# Autodesk Inventor assembly: ASSY,MAIN,ELEVATOR
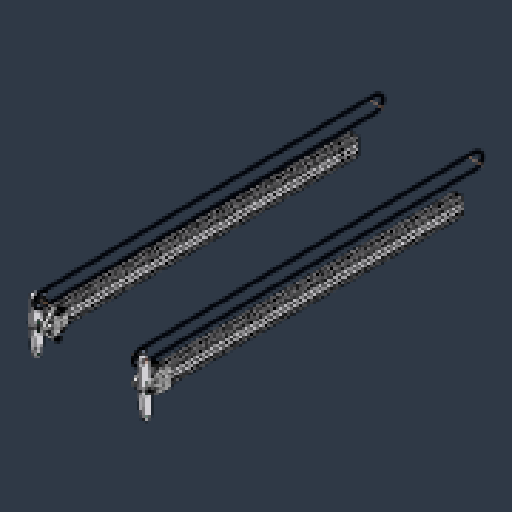
[picture p0: Inventor's stored thumbnail of the model, 512x512]
Saved by Autodesk Inventor 2024.3 (Build 283343000, 343)
## iProperties
Created: 2025-02-06
Part Number: ASSY,MAIN,ELEVATOR
Document SubType Name: Assembly
Designer: Jthib
Mfg Approved By: John.Thibert
Mass: 2913.72 g
Surface Area: 9344.89 cm^2
Volume: 863.068 cm^3
Density: 3.376 g/cm^3
ILogicPurgeVersion: 0.0.0.0
OnSaveVersion: 3.4.3.0
OnSaveAssembly: COREAutomationManager
ModelCat: Uncategorized
CN_MASS: 2.91
Author: Jthib
## Documents named in this file (12)
- C:\Users\Jthib\OneDrive\Robotics\4_Robot Files - 2025 - Poseidon\Elevator\ASSY,MAIN,ELEVATOR.iam
- C:\Users\Jthib\OneDrive\Robotics\4_Robot Files - 2025 - Poseidon\Elevator\SLIDE,TOP,ELEVATOR,STAGE1,LH.iam
- C:\Users\Jthib\OneDrive\Robotics\4_Robot Files - 2025 - Poseidon\Elevator\TUBE,MAIN,ELEVATOR,MAXTube-2x1-Holes.ipt
- C:\Users\Jthib\OneDrive\Robotics\4_Robot Files - 2025 - Poseidon\Chassis\PLUG,MAXTUBE,2IN,3DP.ipt
- C:\Users\Jthib\OneDrive\Robotics\4_Robot Files - 2025 - Poseidon\Elevator\PLUG,MAXTUBE,2IN,3DP,TOP,ELEVATOR.ipt
- C:\Users\Jthib\OneDrive\Robotics\4_Robot Files - 2025 - Poseidon\Elevator\PLATE,SIDE,PULLEY,MOUNT,TOP,ELEVATOR.ipt
- C:\Users\Jthib\OneDrive\Robotics\4_Robot Files - 2025 - Poseidon\Elevator\PLATE,ROCKER,ELEVATOR.ipt
- C:\Users\Jthib\OneDrive\Robotics\4_Robot Files - 2025 - Poseidon\Purchased\6663K11_ANSI Roller Chain Idler Sprocket\6663K11_ANSI Roller Chain Idler Sprocket\6663K11_ANSI Roller Chain Idler Sprocket.ipt
- C:\Users\Jthib\OneDrive\Robotics\4_Robot Files - 2025 - Poseidon\Chassis\#Poseidon 2025\Design Accelerator\Chain Drive2.iam
- C:\Users\Jthib\OneDrive\Robotics\4_Robot Files - 2025 - Poseidon\Elevator\SPACER,ROCKER,ELEVATOR.ipt
- C:\Users\Jthib\OneDrive\Robotics\4_Robot Files - 2025 - Poseidon\Fasteners\91259A585_NO THREADS_Alloy Steel Shoulder Screw\91259A585_NO THREADS_Alloy Steel Shoulder Screw\91259A585_NO THREADS_Alloy Steel Should.ipt
- C:\Users\Jthib\OneDrive\Robotics\4_Robot Files - 2025 - Poseidon\Elevator\SLIDE,TOP,ELEVATOR,STAGE1.iam
## Components (20 placed, 11 different names)
1. 6663K11_ANSI Roller Chain Idler Sprocket.ipt:1 — Mate:46
2. 6663K11_ANSI Roller Chain Idler Sprocket.ipt:2 — Mate:45
3. 91259A585_NO THREADS_Alloy Steel Should.ipt:1
4. 91259A585_NO THREADS_Alloy Steel Should.ipt:2
5. Chain Drive2.iam:1 [sub-assembly] — Mate:43, Mate:44
6. Chain Drive2.iam:2 [sub-assembly] — Mate:44
7. PLATE,ROCKER,ELEVATOR.ipt:1 — Mate:43, Mate:46
8. PLATE,ROCKER,ELEVATOR.ipt:2 — Mate:45
9. PLATE,SIDE,PULLEY,MOUNT,TOP,ELEVATOR.ipt:1
10. PLATE,SIDE,PULLEY,MOUNT,TOP,ELEVATOR.ipt:2 — Angle:3
11. PLUG,MAXTUBE,2IN,3DP,TOP,ELEVATOR.ipt:1
12. PLUG,MAXTUBE,2IN,3DP,TOP,ELEVATOR.ipt:2
13. PLUG,MAXTUBE,2IN,3DP.ipt:1 — Mate:42
14. PLUG,MAXTUBE,2IN,3DP.ipt:2 — Mate:41
15. SLIDE,TOP,ELEVATOR,STAGE1,LH.iam:1 [sub-assembly]
16. SLIDE,TOP,ELEVATOR,STAGE1.iam:1 [sub-assembly]
17. SPACER,ROCKER,ELEVATOR.ipt:1
18. SPACER,ROCKER,ELEVATOR.ipt:2
19. TUBE,MAIN,ELEVATOR,MAXTube-2x1-Holes.ipt:1 — Mate:39, Flush:5
20. TUBE,MAIN,ELEVATOR,MAXTube-2x1-Holes.ipt:2 — Angle:3, Flush:4, Mate:40
## Relationships (54: Mate 46, Flush 5, Angle 3)
- [Flush]: PLUG,MAXTUBE,2IN,3DP.ipt:1 ↔ TUBE,MAIN,ELEVATOR,MAXTube-2x1-Holes.ipt:1
- [Mate]: PLUG,MAXTUBE,2IN,3DP.ipt:1 ↔ TUBE,MAIN,ELEVATOR,MAXTube-2x1-Holes.ipt:1
- [Angle] (0 deg): PLUG,MAXTUBE,2IN,3DP.ipt:1 ↔ TUBE,MAIN,ELEVATOR,MAXTube-2x1-Holes.ipt:1
- [Mate]: SLIDE,TOP,ELEVATOR,STAGE1,LH.iam:1 ↔ TUBE,MAIN,ELEVATOR,MAXTube-2x1-Holes.ipt:1
- [Mate]: SLIDE,TOP,ELEVATOR,STAGE1,LH.iam:1 ↔ TUBE,MAIN,ELEVATOR,MAXTube-2x1-Holes.ipt:1
- [Mate]: SLIDE,TOP,ELEVATOR,STAGE1,LH.iam:1 ↔ TUBE,MAIN,ELEVATOR,MAXTube-2x1-Holes.ipt:1
- [Mate]: PLUG,MAXTUBE,2IN,3DP,TOP,ELEVATOR.ipt:1 ↔ TUBE,MAIN,ELEVATOR,MAXTube-2x1-Holes.ipt:1
- [Mate]: PLATE,SIDE,PULLEY,MOUNT,TOP,ELEVATOR.ipt:1 ↔ TUBE,MAIN,ELEVATOR,MAXTube-2x1-Holes.ipt:1
- [Mate]: PLATE,SIDE,PULLEY,MOUNT,TOP,ELEVATOR.ipt:1 ↔ PLUG,MAXTUBE,2IN,3DP,TOP,ELEVATOR.ipt:1
- [Mate]: PLATE,SIDE,PULLEY,MOUNT,TOP,ELEVATOR.ipt:1 ↔ PLUG,MAXTUBE,2IN,3DP,TOP,ELEVATOR.ipt:1
- [Mate]: PLATE,ROCKER,ELEVATOR.ipt:1 ↔ PLATE,SIDE,PULLEY,MOUNT,TOP,ELEVATOR.ipt:1
- [Mate]: PLATE,ROCKER,ELEVATOR.ipt:1 ↔ PLATE,SIDE,PULLEY,MOUNT,TOP,ELEVATOR.ipt:1
- [Mate]: PLATE,SIDE,PULLEY,MOUNT,TOP,ELEVATOR.ipt:1 ↔ TUBE,MAIN,ELEVATOR,MAXTube-2x1-Holes.ipt:1
- [Mate]: PLUG,MAXTUBE,2IN,3DP,TOP,ELEVATOR.ipt:1 ↔ TUBE,MAIN,ELEVATOR,MAXTube-2x1-Holes.ipt:1
- [Mate]: 6663K11_ANSI Roller Chain Idler Sprocket.ipt:1 ↔ Chain Drive2.iam:1
- [Mate] (0.1905 mm): 6663K11_ANSI Roller Chain Idler Sprocket.ipt:1 ↔ Chain Drive2.iam:1
- [Mate]: 91259A585_NO THREADS_Alloy Steel Should.ipt:1 ↔ SPACER,ROCKER,ELEVATOR.ipt:1
- [Mate]: 91259A585_NO THREADS_Alloy Steel Should.ipt:1 ↔ PLATE,SIDE,PULLEY,MOUNT,TOP,ELEVATOR.ipt:1
- [Mate]: 91259A585_NO THREADS_Alloy Steel Should.ipt:1 ↔ PLATE,ROCKER,ELEVATOR.ipt:1
- [Mate]: PLATE,ROCKER,ELEVATOR.ipt:1 ↔ SPACER,ROCKER,ELEVATOR.ipt:1
- [Flush]: PLUG,MAXTUBE,2IN,3DP.ipt:2 ↔ TUBE,MAIN,ELEVATOR,MAXTube-2x1-Holes.ipt:2
- [Mate]: PLUG,MAXTUBE,2IN,3DP.ipt:2 ↔ TUBE,MAIN,ELEVATOR,MAXTube-2x1-Holes.ipt:2
- [Angle] (0 deg): PLUG,MAXTUBE,2IN,3DP.ipt:2 ↔ TUBE,MAIN,ELEVATOR,MAXTube-2x1-Holes.ipt:2
- [Mate]: SLIDE,TOP,ELEVATOR,STAGE1.iam:1 ↔ TUBE,MAIN,ELEVATOR,MAXTube-2x1-Holes.ipt:2
- [Mate]: SLIDE,TOP,ELEVATOR,STAGE1.iam:1 ↔ TUBE,MAIN,ELEVATOR,MAXTube-2x1-Holes.ipt:2
- [Mate]: SLIDE,TOP,ELEVATOR,STAGE1.iam:1 ↔ TUBE,MAIN,ELEVATOR,MAXTube-2x1-Holes.ipt:2
- [Mate]: SLIDE,TOP,ELEVATOR,STAGE1.iam:1 ↔ TUBE,MAIN,ELEVATOR,MAXTube-2x1-Holes.ipt:2
- [Mate]: PLUG,MAXTUBE,2IN,3DP,TOP,ELEVATOR.ipt:2 ↔ TUBE,MAIN,ELEVATOR,MAXTube-2x1-Holes.ipt:2
- Angle:3 (0 deg): PLATE,SIDE,PULLEY,MOUNT,TOP,ELEVATOR.ipt:2 ↔ TUBE,MAIN,ELEVATOR,MAXTube-2x1-Holes.ipt:2
- [Mate]: PLUG,MAXTUBE,2IN,3DP,TOP,ELEVATOR.ipt:2 ↔ TUBE,MAIN,ELEVATOR,MAXTube-2x1-Holes.ipt:2
- [Mate]: PLATE,SIDE,PULLEY,MOUNT,TOP,ELEVATOR.ipt:2 ↔ TUBE,MAIN,ELEVATOR,MAXTube-2x1-Holes.ipt:2
- [Mate]: PLATE,SIDE,PULLEY,MOUNT,TOP,ELEVATOR.ipt:2 ↔ PLUG,MAXTUBE,2IN,3DP,TOP,ELEVATOR.ipt:2
- [Mate]: PLATE,SIDE,PULLEY,MOUNT,TOP,ELEVATOR.ipt:2 ↔ PLUG,MAXTUBE,2IN,3DP,TOP,ELEVATOR.ipt:2
- [Mate]: PLATE,ROCKER,ELEVATOR.ipt:2 ↔ PLATE,SIDE,PULLEY,MOUNT,TOP,ELEVATOR.ipt:2
- [Mate]: PLATE,ROCKER,ELEVATOR.ipt:2 ↔ PLATE,SIDE,PULLEY,MOUNT,TOP,ELEVATOR.ipt:2
- [Mate]: PLATE,ROCKER,ELEVATOR.ipt:1 ↔ PLATE,ROCKER,ELEVATOR.ipt:2
- [Mate]: 6663K11_ANSI Roller Chain Idler Sprocket.ipt:2 ↔ PLATE,ROCKER,ELEVATOR.ipt:2
- [Mate]: 6663K11_ANSI Roller Chain Idler Sprocket.ipt:2 ↔ Chain Drive2.iam:2
- [Mate] (0.1905 mm): 6663K11_ANSI Roller Chain Idler Sprocket.ipt:2 ↔ Chain Drive2.iam:2
- [Mate]: 6663K11_ANSI Roller Chain Idler Sprocket.ipt:1 ↔ 6663K11_ANSI Roller Chain Idler Sprocket.ipt:2
- [Mate]: 91259A585_NO THREADS_Alloy Steel Should.ipt:2 ↔ PLATE,SIDE,PULLEY,MOUNT,TOP,ELEVATOR.ipt:2
- [Mate]: 91259A585_NO THREADS_Alloy Steel Should.ipt:2 ↔ SLIDE,TOP,ELEVATOR,STAGE1.iam:1
- [Flush]: PLATE,ROCKER,ELEVATOR.ipt:2 ↔ SPACER,ROCKER,ELEVATOR.ipt:2
- [Mate]: 91259A585_NO THREADS_Alloy Steel Should.ipt:2 ↔ SPACER,ROCKER,ELEVATOR.ipt:2
- Mate:39 (139.7 mm): TUBE,MAIN,ELEVATOR,MAXTube-2x1-Holes.ipt:1
- Flush:4 (-139.7 mm): TUBE,MAIN,ELEVATOR,MAXTube-2x1-Holes.ipt:2
- Flush:5: TUBE,MAIN,ELEVATOR,MAXTube-2x1-Holes.ipt:1
- Mate:40: TUBE,MAIN,ELEVATOR,MAXTube-2x1-Holes.ipt:2
- Mate:41: PLUG,MAXTUBE,2IN,3DP.ipt:2
- Mate:42: PLUG,MAXTUBE,2IN,3DP.ipt:1
- Mate:43: Chain Drive2.iam:1 ↔ PLATE,ROCKER,ELEVATOR.ipt:1
- Mate:44: Chain Drive2.iam:1 ↔ Chain Drive2.iam:2
- Mate:45: 6663K11_ANSI Roller Chain Idler Sprocket.ipt:2 ↔ PLATE,ROCKER,ELEVATOR.ipt:2
- Mate:46: 6663K11_ANSI Roller Chain Idler Sprocket.ipt:1 ↔ PLATE,ROCKER,ELEVATOR.ipt:1
## Named parameters: d385_d71 = 0 mm, d386_d72 = 0 mm, d387_d73 = 0 deg
